# Autodesk Inventor assembly: Gimbal
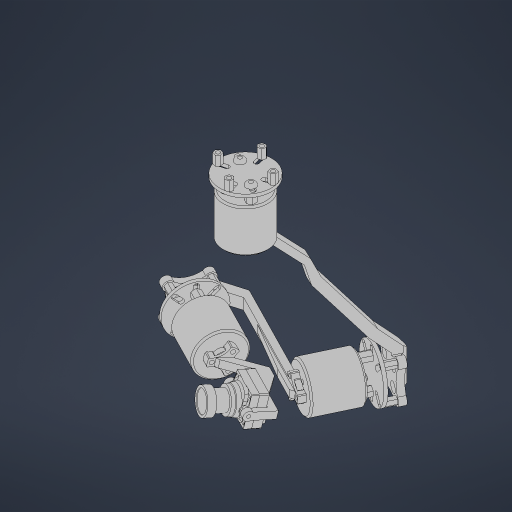
[picture p0: Inventor's stored thumbnail of the model, 512x512]
Saved by Autodesk Inventor 2024.2 (Build 282272000, 272)
## iProperties
Created: 2026-10-01
Part Number: Gimbal
Document SubType Name: Assembly
Designer: Osas
Author: Osas
## Documents named in this file (6)
- C:\Users\Osas\Documents\Project\Подвес\Gimbal.iam
- C:\Users\Osas\Documents\Project\Подвес\CAM.ipt
- C:\Users\Osas\Documents\Project\Подвес\CAM_Hand.ipt
- C:\Users\Osas\Documents\Project\Подвес\BLDC_Gimbal+Enc.ipt
- C:\Users\Osas\Documents\Project\Подвес\BLDC_Hand_1.ipt
- C:\Users\Osas\Documents\Project\Подвес\BLDC_Hand_2.ipt
## Components (7 placed, 5 different names)
1. CAM:1 — Жесткий:1
2. CAM_Hand:1 — Жесткий:1, С поворотом:1, Совмещение:1
3. BLDC_Gimbal+Enc:1 — С поворотом:1, Жесткий:2
4. BLDC_Hand_1:1 — Жесткий:2, С поворотом:2
5. BLDC_Gimbal+Enc:2 — С поворотом:2, Жесткий:3
6. BLDC_Hand_2:1 — Жесткий:3, С поворотом:3
7. BLDC_Gimbal+Enc:3 — С поворотом:3
## Relationships (7: WeldJoint 3, RevoluteJoint 3, Mate 1)
- Жесткий:1 [WeldJoint] (-0.1 mm): CAM:1 ↔ CAM_Hand:1
- С поворотом:1 [RevoluteJoint]: CAM_Hand:1 ↔ BLDC_Gimbal+Enc:1
- Жесткий:2 [WeldJoint]: BLDC_Gimbal+Enc:1 ↔ BLDC_Hand_1:1
- С поворотом:2 [RevoluteJoint]: BLDC_Hand_1:1 ↔ BLDC_Gimbal+Enc:2
- Жесткий:3 [WeldJoint]: BLDC_Gimbal+Enc:2 ↔ BLDC_Hand_2:1
- Совмещение:1 [Mate]: CAM_Hand:1
- С поворотом:3 [RevoluteJoint]: BLDC_Hand_2:1 ↔ BLDC_Gimbal+Enc:3
